# Autodesk Inventor assembly: ShakerAssembly
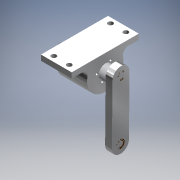
[picture p0: Inventor's stored thumbnail of the model, 180x180]
Saved by Autodesk Inventor 2017 (Build 210142000, 142)
## iProperties
Created: 2017-02-08
Part Number: ShakerAssembly
Document SubType Name: Assembly
Designer: Joseph
Author: Joseph
## Documents named in this file (7)
- C:\UMD\BPP\ROCKSAT X\star\CAD\Mechanical\Full payload assembly\Subsystems\ShakerCAD\ShakerAssembly.iam
- C:\Users\qupec\Desktop\UMD Near Space\RockSat\ShakerCAD\MotorMount.ipt
- C:\UMD\BPP\ROCKSAT X\star\CAD\Mechanical\Full payload assembly\Subsystems\ShakerCAD\Motor.ipt
- C:\UMD\BPP\ROCKSAT X\star\CAD\Mechanical\Full payload assembly\Subsystems\ShakerCAD\Motor Arm.ipt
- C:\UMD\BPP\ROCKSAT X\star\CAD\Mechanical\Full payload assembly\Subsystems\ShakerCAD\Linkage.ipt
- C:\UMD\BPP\ROCKSAT X\star\CAD\Mechanical\Full payload assembly\Subsystems\ShakerCAD\Motor Holder.ipt
- C:\UMD\BPP\ROCKSAT X\star\CAD\Mechanical\Full payload assembly\Subsystems\ShakerCAD\Bearing correct.ipt
## Components (7 placed, 6 different names)
1. MotorMount:1 — Insert:1, Insert:2
2. Motor:1 — Insert:1, Insert:2, Rotational:1, Mate:2, Mate:3, Mate:4, Mate:5
3. Motor Arm:1 — Rotational:1
4. Linkage:1 — Mate:8, Mate:9, Flush:1, Flush:2
5. Motor Holder:1 — Mate:2, Mate:3, Mate:4, Mate:5
6. Bearing correct:1 — Mate:8, Flush:2
7. Bearing correct:2 — Mate:9, Flush:1
## Relationships (11: Mate 6, Insert 2, Flush 2, RevoluteJoint 1)
- Insert:1: MotorMount:1 ↔ Motor:1
- Insert:2: MotorMount:1 ↔ Motor:1
- Rotational:1 [RevoluteJoint]: Motor:1 ↔ Motor Arm:1
- Mate:2: Motor:1 ↔ Motor Holder:1
- Mate:3: Motor:1 ↔ Motor Holder:1
- Mate:4: Motor:1 ↔ Motor Holder:1
- Mate:5: Motor:1 ↔ Motor Holder:1
- Mate:8: Linkage:1 ↔ Bearing correct:1
- Mate:9: Linkage:1 ↔ Bearing correct:2
- Flush:1: Linkage:1 ↔ Bearing correct:2
- Flush:2: Linkage:1 ↔ Bearing correct:1
